# Autodesk Inventor assembly: ГЛАЗ НОВЫЙ СБОРКА
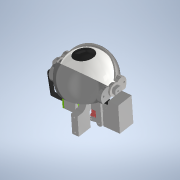
[picture p0: Inventor's stored thumbnail of the model, 180x180]
Saved by Autodesk Inventor 2020 (Build 240168000, 168)
## iProperties
Created: 2022-02-16
Part Number: ГЛАЗ НОВЫЙ СБОРКА
Document SubType Name: Assembly
Designer: Администратор
Author: Администратор
## Documents named in this file (14)
- \\sch239.net\UserHomes\Students\Other\glazovaes\3D\Onstage\Face\ГЛАЗ НОВЫЙ СБОРКА.iam
- \\sch239.net\UserHomes\Students\Other\glazovaes\3D\Onstage\Face\верхнее веко.ipt
- \\sch239.net\UserHomes\Students\Other\glazovaes\3D\Onstage\Face\держалка глаза.ipt
- \\sch239.net\UserHomes\Students\Other\glazovaes\3D\Onstage\Face\шатун движенияглаза.ipt
- \\sch239.net\UserHomes\Students\Other\glazovaes\3D\Onstage\Face\связующий сервы движения глаз.ipt
- \\sch239.net\UserHomes\Students\Other\glazovaes\3D\Onstage\Face\связующий сервы век.ipt
- \\sch239.net\UserHomes\Students\Other\glazovaes\3D\Onstage\Face\нижний шатун век.ipt
- \\sch239.net\UserHomes\Students\Other\glazovaes\3D\Onstage\Face\нижнее веко.ipt
- \\sch239.net\UserHomes\Students\Other\glazovaes\3D\Onstage\Face\держалка сервы движения глаз.ipt
- \\sch239.net\UserHomes\Students\Other\glazovaes\3D\Onstage\Face\держалка сервы век.ipt
- \\sch239.net\UserHomes\Students\Other\glazovaes\3D\Onstage\Face\SERVO.ipt
- \\sch239.net\UserHomes\Students\Other\glazovaes\3D\Onstage\Face\зрачок.ipt
- \\sch239.net\UserHomes\Students\Other\glazovaes\3D\Onstage\Face\белок глаза_ЗЕРКАЛО.ipt
- \\sch239.net\UserHomes\Students\Other\glazovaes\3D\Onstage\Face\верхний шатун века_ЗЕРКАЛО1.ipt
## Components (14 placed, 13 different names)
1. шатун движенияглаза:1 — Совмещение:30, Совмещение:31, Совмещение:46, Совмещение:47
2. связующий сервы движения глаз:1 — Совмещение:16, Совмещение:20, Совмещение:43, Совмещение:44
3. связующий сервы век:1 — Совмещение:30, Совмещение:31, Совмещение:38
4. верхнее веко — Совмещение:5, Совмещение:6, Совмещение:7, Совмещение:8, Совмещение:9, Совмещение:41, Совмещение:42
5. держалка сервы движения глаз:1 — Совмещение:32, Совмещение:33, Совмещение:34, Совмещение:35, Совмещение:36, Совмещение:37
6. держалка сервы век:1 — Совмещение:21, Совмещение:22, Совмещение:23
7. держалка глаза:1 — Совмещение:5, Совмещение:6, Совмещение:7, Совмещение:10, Совмещение:18, Совмещение:19, Угол:1, Совмещение:32, Совмещение:33, Совмещение:34, Совмещение:45, Совмещение:48
8. нижнее веко — Совмещение:8, Совмещение:9, Совмещение:10, Совмещение:13, Совмещение:14
9. SERVO:1 — Совмещение:18, Совмещение:19, Угол:1, Совмещение:20, Совмещение:21, Совмещение:22, Совмещение:23, Совмещение:43
10. SERVO:2 — Совмещение:35, Совмещение:36, Совмещение:37, Совмещение:38
11. нижний шатун век:1 — Совмещение:13, Совмещение:14, Совмещение:16
12. зрачок:1 — Совмещение:39, Совмещение:40
13. белок глаза_ЗЕРКАЛО:2 — Совмещение:39, Совмещение:40, Совмещение:45, Совмещение:46, Совмещение:47, Совмещение:48
14. верхний шатун века_ЗЕРКАЛО1:1 — Совмещение:41, Совмещение:42, Совмещение:44
## Relationships (35: Mate 34, Angle 1)
- Совмещение:5 [Mate]: верхнее веко ↔ держалка глаза:1
- Совмещение:6 [Mate]: верхнее веко ↔ держалка глаза:1
- Совмещение:7 [Mate]: верхнее веко ↔ держалка глаза:1
- Совмещение:8 [Mate]: верхнее веко ↔ нижнее веко
- Совмещение:9 [Mate]: верхнее веко ↔ нижнее веко
- Совмещение:10 [Mate]: держалка глаза:1 ↔ нижнее веко
- Совмещение:13 [Mate]: нижнее веко ↔ нижний шатун век:1
- Совмещение:14 [Mate]: нижнее веко ↔ нижний шатун век:1
- Совмещение:16 [Mate]: связующий сервы движения глаз:1 ↔ нижний шатун век:1
- Совмещение:18 [Mate]: держалка глаза:1 ↔ SERVO:1
- Совмещение:19 [Mate]: держалка глаза:1 ↔ SERVO:1
- Угол:1 [Angle] (0 deg): держалка глаза:1 ↔ SERVO:1
- Совмещение:20 [Mate]: связующий сервы движения глаз:1 ↔ SERVO:1
- Совмещение:21 [Mate]: держалка сервы век:1 ↔ SERVO:1
- Совмещение:22 [Mate]: держалка сервы век:1 ↔ SERVO:1
- Совмещение:23 [Mate]: держалка сервы век:1 ↔ SERVO:1
- Совмещение:30 [Mate]: шатун движенияглаза:1 ↔ связующий сервы век:1
- Совмещение:31 [Mate]: шатун движенияглаза:1 ↔ связующий сервы век:1
- Совмещение:32 [Mate]: держалка сервы движения глаз:1 ↔ держалка глаза:1
- Совмещение:33 [Mate]: держалка сервы движения глаз:1 ↔ держалка глаза:1
- Совмещение:34 [Mate]: держалка сервы движения глаз:1 ↔ держалка глаза:1
- Совмещение:35 [Mate]: держалка сервы движения глаз:1 ↔ SERVO:2
- Совмещение:36 [Mate]: держалка сервы движения глаз:1 ↔ SERVO:2
- Совмещение:37 [Mate]: держалка сервы движения глаз:1 ↔ SERVO:2
- Совмещение:38 [Mate]: связующий сервы век:1 ↔ SERVO:2
- Совмещение:39 [Mate]: зрачок:1 ↔ белок глаза_ЗЕРКАЛО:2
- Совмещение:40 [Mate]: зрачок:1 ↔ белок глаза_ЗЕРКАЛО:2
- Совмещение:41 [Mate]: верхнее веко ↔ верхний шатун века_ЗЕРКАЛО1:1
- Совмещение:42 [Mate]: верхнее веко ↔ верхний шатун века_ЗЕРКАЛО1:1
- Совмещение:43 [Mate]: связующий сервы движения глаз:1 ↔ SERVO:1
- Совмещение:44 [Mate]: связующий сервы движения глаз:1 ↔ верхний шатун века_ЗЕРКАЛО1:1
- Совмещение:45 [Mate]: держалка глаза:1 ↔ белок глаза_ЗЕРКАЛО:2
- Совмещение:46 [Mate]: шатун движенияглаза:1 ↔ белок глаза_ЗЕРКАЛО:2
- Совмещение:47 [Mate]: шатун движенияглаза:1 ↔ белок глаза_ЗЕРКАЛО:2
- Совмещение:48 [Mate]: держалка глаза:1 ↔ белок глаза_ЗЕРКАЛО:2
